# Autodesk Inventor assembly: Assembly1
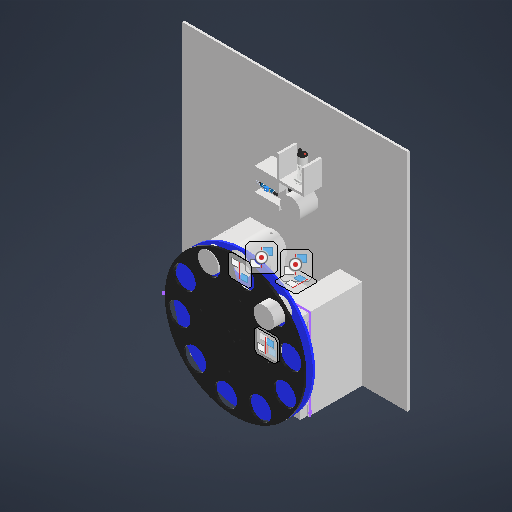
[picture p0: Inventor's stored thumbnail of the model, 512x512]
Saved by Autodesk Inventor 2027.1 (Build 311270010, 270A)
## iProperties
Created: 2026-09-28
Part Number: Assembly1
Document SubType Name: Assembly
Designer: daniel
Author: daniel
## Documents named in this file (14)
- C:\Users\danda\Documents\GitHub\MCT333_Design_of_Mechatronics_Systems_1\CAD\FEED and Sorting\Assembly1.iam
- C:\Users\danda\Documents\GitHub\MCT333_Design_of_Mechatronics_Systems_1\CAD\FEED and Sorting\Part2.ipt
- C:\Users\danda\Documents\GitHub\MCT333_Design_of_Mechatronics_Systems_1\CAD\FEED and Sorting\Part1.ipt
- C:\Users\danda\Documents\GitHub\MCT333_Design_of_Mechatronics_Systems_1\CAD\FEED and Sorting\base.ipt
- C:\Users\danda\Documents\GitHub\MCT333_Design_of_Mechatronics_Systems_1\CAD\off_the_shelf_components\standard-servo-motor-black-1.snapshot.7\Assem1\Assem1.iam
- C:\Users\danda\Documents\GitHub\MCT333_Design_of_Mechatronics_Systems_1\CAD\FEED and Sorting\Part22.ipt
- C:\Users\danda\Documents\GitHub\MCT333_Design_of_Mechatronics_Systems_1\CAD\FEED and Sorting\Part23.ipt
- C:\Users\danda\Documents\GitHub\MCT333_Design_of_Mechatronics_Systems_1\CAD\FEED and Sorting\Part24.ipt
- C:\Users\danda\Documents\GitHub\MCT333_Design_of_Mechatronics_Systems_1\CAD\FEED and Sorting\Assembly7.iam
- C:\Users\danda\Documents\GitHub\MCT333_Design_of_Mechatronics_Systems_1\CAD\FEED and Sorting\Part27.ipt
- C:\Users\danda\Documents\GitHub\MCT333_Design_of_Mechatronics_Systems_1\CAD\FEED and Sorting\box\Assembly1.iam
- C:\Users\danda\Documents\GitHub\MCT333_Design_of_Mechatronics_Systems_1\CAD\FEED and Sorting\Part67.ipt
- C:\Users\danda\Documents\Inventor\Content Center Files\R2027\en-US\GB_T 301-1995(51000)\Rolling bearing 51109 GB_T 301-1995.ipt
- C:\Users\danda\Documents\GitHub\MCT333_Design_of_Mechatronics_Systems_1\CAD\FEED and Sorting\Part69.ipt
## Components (14 placed, 13 different names)
1. Part2:1 — Tangent:1, Tangent:2, Mate:42, Mate:43, Mate:44, Mate:45, Mate:46
2. Part1:1 — Mate:8, Mate:9, Mate:15, Mate:16, Mate:34, Mate:36, Mate:37, Mate:38, Mate:40, Mate:41
3. base:1 — Mate:19, Flush:21, Mate:20, Mate:21, Flush:22, Flush:23
4. Assem1:1 [sub-assembly] — Mate:22, Mate:23, Mate:28, Mate:29, Mate:30, Mate:37, Mate:39, Mate:42, Mate:43, Mate:44
5. Part22:1 — Mate:8, Mate:9
6. Part23:1 — Tangent:1, Mate:15
7. Part24:1 — Mate:16, Tangent:2
8. Assembly7:1 [sub-assembly] — Mate:19, Flush:21
9. Part27:1 — Flush:24, Mate:33, Mate:34
10. Assembly1:1 [sub-assembly] — Mate:20, Mate:21, Flush:22, Flush:23, Mate:22, Mate:23, Mate:28, Mate:29, Mate:30, Flush:24, Mate:33, Flush:25, Flush:26, Mate:35
11. Part67:1 — Flush:25, Flush:26, Mate:35, Mate:36
12. Rolling bearing GB/T 301-1995 Type 51000 51109:1 — Mate:38, Mate:39, Tangent:3, Tangent:4
13. Part69:1 — Mate:40, Mate:41, Tangent:3
14. Part69:2 — Tangent:4, Mate:45, Mate:46
## Relationships (36: Mate 26, Flush 6, Tangent 4)
- Mate:8: Part1:1 ↔ Part22:1
- Mate:9: Part1:1 ↔ Part22:1
- Tangent:1: Part2:1 ↔ Part23:1
- Mate:15: Part1:1 ↔ Part23:1
- Mate:16: Part1:1 ↔ Part24:1
- Tangent:2: Part2:1 ↔ Part24:1
- Mate:19: base:1 ↔ Assembly7:1
- Flush:21 (190 mm): base:1 ↔ Assembly7:1
- Mate:20: base:1 ↔ Assembly1:1
- Mate:21: base:1 ↔ Assembly1:1
- Flush:22: base:1 ↔ Assembly1:1
- Flush:23 (100 mm): base:1 ↔ Assembly1:1
- Mate:22: Assem1:1 ↔ Assembly1:1
- Mate:23: Assem1:1 ↔ Assembly1:1
- Mate:28: Assem1:1 ↔ Assembly1:1
- Mate:29: Assem1:1 ↔ Assembly1:1
- Mate:30: Assem1:1 ↔ Assembly1:1
- Flush:24: Part27:1 ↔ Assembly1:1
- Mate:33: Part27:1 ↔ Assembly1:1
- Mate:34: Part1:1 ↔ Part27:1
- Flush:25: Assembly1:1 ↔ Part67:1
- Flush:26: Assembly1:1 ↔ Part67:1
- Mate:35: Assembly1:1 ↔ Part67:1
- Mate:36: Part1:1 ↔ Part67:1
- Mate:37: Part1:1 ↔ Assem1:1
- Mate:38: Part1:1 ↔ Rolling bearing GB/T 301-1995 Type 51000 51109:1
- Mate:39: Assem1:1 ↔ Rolling bearing GB/T 301-1995 Type 51000 51109:1
- Mate:40: Part1:1 ↔ Part69:1
- Mate:41: Part1:1 ↔ Part69:1
- Tangent:3: Rolling bearing GB/T 301-1995 Type 51000 51109:1 ↔ Part69:1
- Mate:42: Part2:1 ↔ Assem1:1
- Mate:43: Part2:1 ↔ Assem1:1
- Mate:44: Part2:1 ↔ Assem1:1
- Tangent:4: Rolling bearing GB/T 301-1995 Type 51000 51109:1 ↔ Part69:2
- Mate:45: Part2:1 ↔ Part69:2
- Mate:46: Part2:1 ↔ Part69:2
